# Autodesk Inventor assembly: Assembly3
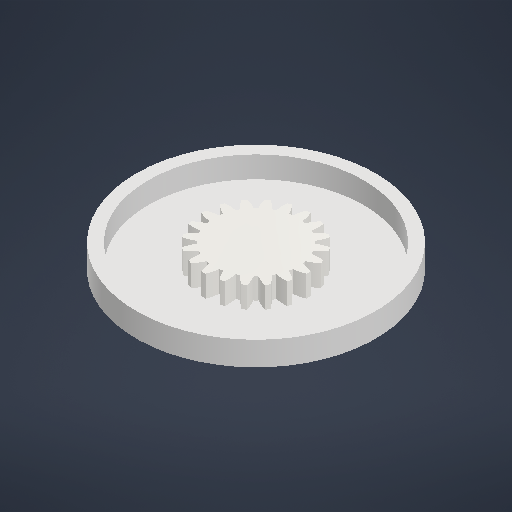
[picture p0: Inventor's stored thumbnail of the model, 512x512]
Saved by Autodesk Inventor 2027.1 (Build 311267000, 267)
## iProperties
Created: 2026-10-02
Part Number: Assembly3
Document SubType Name: Assembly
Designer: HP
Author: HP
## Documents named in this file (3)
- C:\Users\HP\Documents\GitHub\Robotic-arm\3dfiles\Assembly3.iam
- C:\Users\HP\Documents\GitHub\Robotic-arm\3dfiles\Gearsp1.ipt
- C:\Users\HP\Documents\GitHub\Robotic-arm\3dfiles\Assembly3\Design Accelerator\Spur Gears5.iam
## Components (2 placed, 2 different names)
1. Gearsp1:1 — Mate:1, Mate:2
2. Spur Gears:1 [sub-assembly] — Mate:1, Mate:2
## Relationships (2: Mate 2)
- Mate:1: Gearsp1:1 ↔ Spur Gears:1
- Mate:2: Gearsp1:1 ↔ Spur Gears:1
